# Autodesk Inventor assembly: BS_Assembly_Coupled_BSAdapterV9
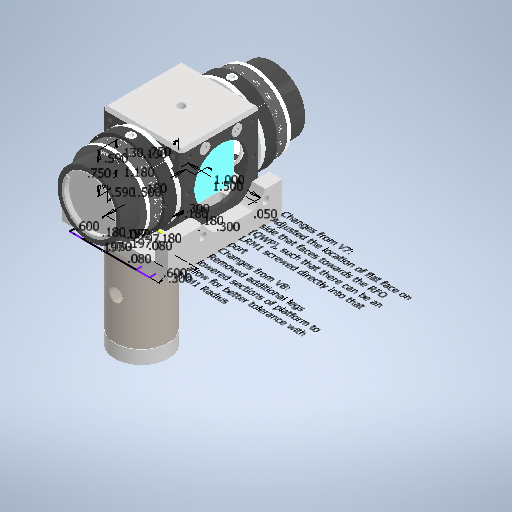
[picture p0: Inventor's stored thumbnail of the model, 512x512]
Saved by Autodesk Inventor 2025.2 (Build 292293000, 293)
## iProperties
Created: 2025-10-27
Part Number: BS_Assembly_Coupled_BSAdapterV9
Document SubType Name: Assembly
Designer: monolithic
Author: monolithic
## Documents named in this file (8)
- C:\Users\monolithic\Documents\GitHub\CAD\Monolith\John\Altair_PowellAndCylindricalBaseplatesCombined_10_16_2025\Assemblies\Subassemblies\BS_Assembly_Coupled_BSAdapterV9.iam
- C:\Users\monolithic\Documents\GitHub\CAD\Monolith\John\Altair_PowellBaseplate_SPIM_ASLM_CTASLM\Assembly\SubAssemblies\PLS-P150.ipt
- C:\Users\monolithic\Documents\GitHub\CAD\Monolith\John\Altair_PowellBaseplate_SPIM_ASLM_CTASLM\Assembly\SubAssemblies\CCM1-WPBS254_M-Step.ipt
- C:\Users\monolithic\Documents\GitHub\CAD\Monolith\John\PolarisPost_HeightAdjustment_0p25in_smallholesfrom0p79to0p81.ipt
- C:\Users\monolithic\Documents\GitHub\CAD\Monolith\John\Altair_PowellBaseplate_SPIM_ASLM_CTASLM\Assembly\SubAssemblies\LRM1-Step.ipt
- C:\Users\monolithic\Documents\GitHub\CAD\Monolith\John\Altair_PowellBaseplate_SPIM_ASLM_CTASLM\Assembly\SubAssemblies\AHWP10M-580-Step.ipt
- C:\Users\monolithic\Documents\GitHub\CAD\Monolith\John\Altair_PowellAndCylindricalBaseplatesCombined_10_16_2025\Assemblies\Subassemblies\P25K1-Step\P25K1-Step\P25K1-Step.iam
- C:\Users\monolithic\Documents\GitHub\CAD\Monolith\John\BeamsplitterMounttoPolarisPinAdapterV9.ipt
## Components (9 placed, 7 different names)
1. PLS-P150:1 — Mate:6, Mate:7, Mate:21, Mate:26
2. CCM1-WPBS254_M-Step:1 — Angle:1, Mate:8, Mate:9, Mate:13, Angle:2, Mate:14, Mate:17, Mate:18, Mate:23, Mate:24, Mate:25
3. PolarisPost_HeightAdjustment_0p25in_smallholesfrom0p79to0p81:1 — Mate:6, Mate:7
4. LRM1-Step:1 — Angle:1, Mate:8, Mate:9, Mate:10, Mate:19
5. AHWP10M-580-Step:1 — Mate:10, Mate:19
6. LRM1-Step:2 — Mate:13, Angle:2, Mate:14, Mate:15, Mate:16
7. AHWP10M-580-Step:2 — Mate:15, Mate:16
8. P25K1-Step:1 [sub-assembly] — Mate:17, Mate:18
9. BeamsplitterMounttoPolarisPinAdapterV9:1 — Mate:21, Mate:23, Mate:24, Mate:25, Mate:26
## Relationships (19: Mate 17, Angle 2)
- Mate:6: PLS-P150:1 ↔ PolarisPost_HeightAdjustment_0p25in_smallholesfrom0p79to0p81:1
- Mate:7: PLS-P150:1 ↔ PolarisPost_HeightAdjustment_0p25in_smallholesfrom0p79to0p81:1
- Angle:1 (0 deg): CCM1-WPBS254_M-Step:1 ↔ LRM1-Step:1
- Mate:8: CCM1-WPBS254_M-Step:1 ↔ LRM1-Step:1
- Mate:9: CCM1-WPBS254_M-Step:1 ↔ LRM1-Step:1
- Mate:10: LRM1-Step:1 ↔ AHWP10M-580-Step:1
- Mate:13: CCM1-WPBS254_M-Step:1 ↔ LRM1-Step:2
- Angle:2 (0 deg): CCM1-WPBS254_M-Step:1 ↔ LRM1-Step:2
- Mate:14: CCM1-WPBS254_M-Step:1 ↔ LRM1-Step:2
- Mate:15: LRM1-Step:2 ↔ AHWP10M-580-Step:2
- Mate:16: LRM1-Step:2 ↔ AHWP10M-580-Step:2
- Mate:17: CCM1-WPBS254_M-Step:1 ↔ P25K1-Step:1
- Mate:18: CCM1-WPBS254_M-Step:1 ↔ P25K1-Step:1
- Mate:19: LRM1-Step:1 ↔ AHWP10M-580-Step:1
- Mate:21: PLS-P150:1 ↔ BeamsplitterMounttoPolarisPinAdapterV9:1
- Mate:23: CCM1-WPBS254_M-Step:1 ↔ BeamsplitterMounttoPolarisPinAdapterV9:1
- Mate:24: CCM1-WPBS254_M-Step:1 ↔ BeamsplitterMounttoPolarisPinAdapterV9:1
- Mate:25: CCM1-WPBS254_M-Step:1 ↔ BeamsplitterMounttoPolarisPinAdapterV9:1
- Mate:26: PLS-P150:1 ↔ BeamsplitterMounttoPolarisPinAdapterV9:1
